# Autodesk Inventor assembly: Assembly
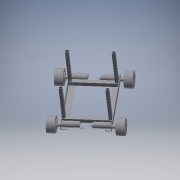
[picture p0: Inventor's stored thumbnail of the model, 180x180]
Saved by Autodesk Inventor 2016 (Build 200138000, 138)
## iProperties
Created: 2017-11-01
Part Number: Assembly
Document SubType Name: Assembly
Designer: thompson.nathaniel
Author: thompson.nathaniel
## Documents named in this file (8)
- \\fs1\studentusers\class18\Thompson.Nathaniel\Documents\Engineering\Robot Assembly\Assembly.iam
- \\fs1\studentusers\class18\Thompson.Nathaniel\Documents\Engineering\Robot Assembly\Cross bar1.ipt
- \\fs1\studentusers\class18\Thompson.Nathaniel\Documents\Engineering\Robot Assembly\Side bar1.ipt
- \\fs1\studentusers\class18\Thompson.Nathaniel\Documents\Engineering\Robot Assembly\Side bar2.ipt
- \\fs1\studentusers\class18\Thompson.Nathaniel\Documents\Engineering\Downloaded parts\REV-41-1301.ipt
- \\fs1\studentusers\class18\Thompson.Nathaniel\Documents\Engineering\Robot Assembly\Motor hub.ipt
- \\fs1\studentusers\class18\Thompson.Nathaniel\Documents\Engineering\Robot Assembly\Simple Wheel.ipt
- \\fs1\studentusers\class18\Thompson.Nathaniel\Documents\Engineering\Robot Assembly\Main upright.ipt
## Components (20 placed, 7 different names)
1. Cross bar1:1 — Mate:1, Mate:2, Flush:1, Mate:8, Flush:4, Mate:36, Mate:37, Flush:7, Flush:8
2. Side bar1:1 — Mate:1, Mate:2, Flush:1, Mate:6, Mate:7, Flush:3, Mate:19, Mate:21, Angle:2, Mate:24, Mate:25, Angle:4, Mate:39, Mate:40
3. Cross bar1:2 — Mate:6, Mate:7, Flush:3, Mate:9, Mate:35, Mate:38, Flush:5, Flush:6
4. Side bar2:1 — Mate:8, Mate:9, Flush:4, Mate:18, Angle:1, Mate:22, Mate:23, Mate:26, Angle:3, Mate:41, Mate:42
5. REV-41-1301:1 — Mate:10, Mate:16, Angle:2
6. REV-41-1301:2 — Mate:11, Mate:15, Angle:3, Mate:30
7. REV-41-1301:3 — Mate:14, Mate:18, Angle:1, Mate:20
8. REV-41-1301:4 — Mate:13, Mate:17, Angle:4
9. Motor hub:1 — Mate:10, Mate:16, Mate:19, Mate:21, Mate:28, Mate:32
10. Motor hub:2 — Mate:14, Mate:20, Mate:22, Mate:27, Mate:31
11. Motor hub:3 — Mate:13, Mate:17, Mate:24, Mate:25, Mate:29, Mate:34
12. Motor hub:4 — Mate:11, Mate:15, Mate:23, Mate:26, Mate:33
13. Simple Wheel:1 — Mate:28, Mate:32
14. Simple Wheel:2 — Mate:29, Mate:34
15. Simple Wheel:3 — Mate:30, Mate:33
16. Simple Wheel:4 — Mate:27, Mate:31
17. Main upright:1 — Mate:38, Mate:39, Flush:5
18. Main upright:2 — Mate:37, Mate:41, Flush:7
19. Main upright:3 — Mate:36, Mate:40, Flush:8
20. Main upright:4 — Mate:35, Mate:42, Flush:6
## Relationships (49: Mate 38, Flush 7, Angle 4)
- Mate:1: Cross bar1:1 ↔ Side bar1:1
- Mate:2: Cross bar1:1 ↔ Side bar1:1
- Flush:1 (44.704 mm): Cross bar1:1 ↔ Side bar1:1
- Mate:6: Side bar1:1 ↔ Cross bar1:2
- Mate:7: Side bar1:1 ↔ Cross bar1:2
- Flush:3 (54.864 mm): Side bar1:1 ↔ Cross bar1:2
- Mate:8: Cross bar1:1 ↔ Side bar2:1
- Mate:9: Cross bar1:2 ↔ Side bar2:1
- Flush:4 (-44.704 mm): Cross bar1:1 ↔ Side bar2:1
- Mate:10: REV-41-1301:1 ↔ Motor hub:1
- Mate:11: REV-41-1301:2 ↔ Motor hub:4
- Mate:13: REV-41-1301:4 ↔ Motor hub:3
- Mate:14: REV-41-1301:3 ↔ Motor hub:2
- Mate:15: REV-41-1301:2 ↔ Motor hub:4
- Mate:16: REV-41-1301:1 ↔ Motor hub:1
- Mate:17: REV-41-1301:4 ↔ Motor hub:3
- Mate:18: Side bar2:1 ↔ REV-41-1301:3
- Angle:1 (180 deg): Side bar2:1 ↔ REV-41-1301:3
- Mate:19: Side bar1:1 ↔ Motor hub:1
- Mate:20: REV-41-1301:3 ↔ Motor hub:2
- Mate:21 (0.254 mm): Side bar1:1 ↔ Motor hub:1
- Angle:2 (180 deg): Side bar1:1 ↔ REV-41-1301:1
- Mate:22 (0.254 mm): Side bar2:1 ↔ Motor hub:2
- Mate:23: Side bar2:1 ↔ Motor hub:4
- Mate:24: Side bar1:1 ↔ Motor hub:3
- Mate:25 (0.254 mm): Side bar1:1 ↔ Motor hub:3
- Mate:26 (0.254 mm): Side bar2:1 ↔ Motor hub:4
- Angle:3 (180 deg): Side bar2:1 ↔ REV-41-1301:2
- Angle:4 (180 deg): Side bar1:1 ↔ REV-41-1301:4
- Mate:27: Motor hub:2 ↔ Simple Wheel:4
- Mate:28: Motor hub:1 ↔ Simple Wheel:1
- Mate:29: Motor hub:3 ↔ Simple Wheel:2
- Mate:30: REV-41-1301:2 ↔ Simple Wheel:3
- Mate:31: Motor hub:2 ↔ Simple Wheel:4
- Mate:32: Motor hub:1 ↔ Simple Wheel:1
- Mate:33: Motor hub:4 ↔ Simple Wheel:3
- Mate:34: Motor hub:3 ↔ Simple Wheel:2
- Mate:35: Cross bar1:2 ↔ Main upright:4
- Mate:36: Cross bar1:1 ↔ Main upright:3
- Mate:37: Cross bar1:1 ↔ Main upright:2
- Mate:38: Cross bar1:2 ↔ Main upright:1
- Mate:39: Side bar1:1 ↔ Main upright:1
- Mate:40: Side bar1:1 ↔ Main upright:3
- Mate:41: Side bar2:1 ↔ Main upright:2
- Mate:42: Side bar2:1 ↔ Main upright:4
- Flush:5 (3.0734 mm): Cross bar1:2 ↔ Main upright:1
- Flush:6 (3.0734 mm): Cross bar1:2 ↔ Main upright:4
- Flush:7 (3.0734 mm): Cross bar1:1 ↔ Main upright:2
- Flush:8 (3.0734 mm): Cross bar1:1 ↔ Main upright:3
